# Autodesk Inventor assembly: end effector worm gear 2
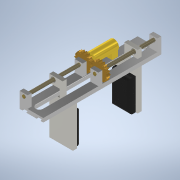
[picture p0: Inventor's stored thumbnail of the model, 180x180]
Saved by Autodesk Inventor 2020 (Build 240168000, 168)
## iProperties
Created: 2020-07-02
Part Number: end effector worm gear 2
Document SubType Name: Assembly
Designer: Ashiqrahman
Author: Ashiqrahman
## Documents named in this file (8)
- D:\projects\Intelligent Picking\end effector worm gear 2.iam
- C:\Users\Public\Documents\Autodesk\Inventor 2020\base plate.ipt
- C:\Users\Public\Documents\Autodesk\Inventor 2020\lead screw.ipt
- C:\Users\Public\Documents\Autodesk\Inventor 2020\lead screw 160.ipt
- D:\projects\Intelligent Picking\end effector worm gear 2\Design Accelerator\Spur Gears2.iam
- C:\Users\Public\Documents\Autodesk\Inventor 2020\jaws.ipt
- C:\Users\Public\Documents\Autodesk\Inventor 2020\motor jaws.ipt
- C:\Users\Public\Documents\Autodesk\Inventor 2020\rubber padding.ipt
## Components (9 placed, 7 different names)
1. base plate:1 — Mate:1, Flush:1, Mate:2, Flush:2, Flush:3, Mate:8
2. lead screw:1 — Mate:2, Flush:2, Mate:3, Mate:5, Mate:7, Rotation/Translation:2
3. lead screw 160:1 — Mate:1, Flush:1, Mate:4, Mate:6, Rotation/Translation:1, Flush:4
4. Spur Gears:2 [sub-assembly] — Mate:3, Mate:4, Flush:3, Mate:5, Mate:6
5. jaws:1 — Rotation/Translation:1, Mate:10, Flush:12, Flush:13
6. jaws:2 — Mate:7, Mate:8, Rotation/Translation:2, Flush:5, Mate:9, Flush:6, Flush:7
7. motor jaws:1 — Flush:4
8. rubber padding:1 — Flush:5, Mate:9, Flush:6, Flush:7
9. rubber padding:2 — Mate:10, Flush:12, Flush:13
## Relationships (21: Mate 10, Flush 9, RelateRotateTranslate 2)
- Mate:1: base plate:1 ↔ lead screw 160:1
- Flush:1: base plate:1 ↔ lead screw 160:1
- Mate:2: base plate:1 ↔ lead screw:1
- Flush:2: base plate:1 ↔ lead screw:1
- Mate:3: lead screw:1 ↔ Spur Gears:2
- Mate:4: lead screw 160:1 ↔ Spur Gears:2
- Flush:3 (11 mm): base plate:1 ↔ Spur Gears:2
- Mate:5: lead screw:1 ↔ Spur Gears:2
- Mate:6: lead screw 160:1 ↔ Spur Gears:2
- Mate:7: lead screw:1 ↔ jaws:2
- Mate:8: base plate:1 ↔ jaws:2
- Rotation/Translation:1 [RelateRotateTranslate] (25.133 mm): lead screw 160:1 ↔ jaws:1
- Rotation/Translation:2 [RelateRotateTranslate] (25.133 mm): lead screw:1 ↔ jaws:2
- Flush:4: lead screw 160:1 ↔ motor jaws:1
- Flush:5: jaws:2 ↔ rubber padding:1
- Mate:9: jaws:2 ↔ rubber padding:1
- Flush:6 (5 mm): jaws:2 ↔ rubber padding:1
- Flush:7: jaws:2 ↔ rubber padding:1
- Mate:10: jaws:1 ↔ rubber padding:2
- Flush:12: jaws:1 ↔ rubber padding:2
- Flush:13 (5 mm): jaws:1 ↔ rubber padding:2
